# Autodesk Inventor assembly: Z Axis
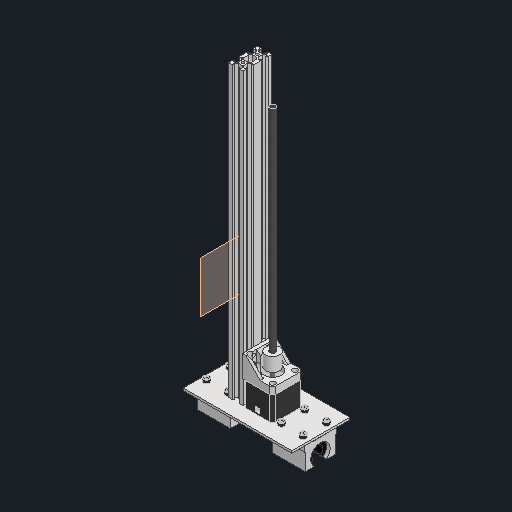
[picture p0: Inventor's stored thumbnail of the model, 512x512]
Saved by Autodesk Inventor 2025.1 (Build 291241000, 241)
## iProperties
Created: 2025-01-21
Part Number: Z Axis
Document SubType Name: Assembly
Designer: jerem
Author: jerem
## Documents named in this file (10)
- C:\Users\jerem\Documents\GitHub\Perovskite-Automated-Synthesis-System\CAD\Gantry\Z Axis.iam
- C:\Users\jerem\Documents\GitHub\Perovskite-Automated-Synthesis-System\CAD\Non 3D Printed Parts\X Axis Base Plate.ipt
- C:\Users\jerem\Documents\GitHub\Perovskite-Automated-Synthesis-System\CAD\Non 3D Printed Parts\Extrusion\V Extrustion 40x400mm.ipt
- C:\Users\jerem\Documents\GitHub\Perovskite-Automated-Synthesis-System\CAD\Non 3D Printed Parts\Screws\M5x12.ipt
- C:\Users\jerem\Documents\GitHub\Perovskite-Automated-Synthesis-System\CAD\Non 3D Printed Parts\Motors and Servos\NEMA17 Stepper Motor.ipt
- C:\Users\jerem\Documents\GitHub\Perovskite-Automated-Synthesis-System\CAD\Non 3D Printed Parts\Threaded Rod 300mm.ipt
- C:\Users\jerem\Documents\GitHub\Perovskite-Automated-Synthesis-System\CAD\Non 3D Printed Parts\Rod Coupler.ipt
- C:\Users\jerem\Documents\GitHub\Perovskite-Automated-Synthesis-System\CAD\Non 3D Printed Parts\Nuts\M4 T-Slot Nut.ipt
- C:\Users\jerem\Documents\GitHub\Perovskite-Automated-Synthesis-System\CAD\Gantry\Z Axis Motor Mount.ipt
- C:\Users\jerem\Documents\GitHub\Perovskite-Automated-Synthesis-System\CAD\Non 3D Printed Parts\Linear Rails\Linear Rail Slider Block.ipt
## Components (18 placed, 9 different names)
1. X Axis Base Plate:1 — Mate:1, Mate:2, Mate:3, Mate:4, Mate:5, Mate:6, Mate:7, Mate:8, Mate:9, Mate:10, Mate:11, Mate:12, Mate:13, Mate:14, Mate:15, Mate:16, Mate:17, Mate:26, Angle:1, Flush:2, Mate:42, Mate:43
2. V Extrustion 40x400mm:1 — Mate:1, Mate:25, Angle:1, Mate:30, Angle:2, Angle:3, Mate:32, Flush:1, Tangent:1
3. M5x12:1 — Mate:2, Mate:3, Mate:47
4. M5x12:2 — Mate:4, Mate:17
5. M5x12:3 — Mate:9, Mate:12
6. M5x12:4 — Mate:8, Mate:13
7. M5x12:5 — Mate:7, Mate:15, Tangent:1
8. M5x12:6 — Mate:6, Mate:14, Mate:45
9. M5x12:7 — Mate:5, Mate:16, Mate:46
10. M5x12:8 — Mate:10, Mate:11, Mate:44
11. NEMA17 Stepper Motor:1 — Mate:25, Mate:26, Mate:33, Mate:34, Mate:35, Flush:1, Flush:2
12. Threaded Rod 300mm:1
13. Rod Coupler:1
14. M4 T-Slot Nut:1 — Mate:30, Angle:2, Mate:37
15. M4 T-Slot Nut:2 — Angle:3, Mate:32, Mate:36
16. Z Axis Motor Mount:1 — Mate:33, Mate:34, Mate:35, Mate:36, Mate:37
17. Linear Rail Slider Block:1 — Mate:43, Mate:44, Mate:45
18. Linear Rail Slider Block:2 — Mate:42, Mate:46, Mate:47
## Relationships (42: Mate 36, Angle 3, Flush 2, Tangent 1)
- Mate:1: X Axis Base Plate:1 ↔ V Extrustion 40x400mm:1
- Mate:2: X Axis Base Plate:1 ↔ M5x12:1
- Mate:3: X Axis Base Plate:1 ↔ M5x12:1
- Mate:4: X Axis Base Plate:1 ↔ M5x12:2
- Mate:5: X Axis Base Plate:1 ↔ M5x12:7
- Mate:6: X Axis Base Plate:1 ↔ M5x12:6
- Mate:7: X Axis Base Plate:1 ↔ M5x12:5
- Mate:8: X Axis Base Plate:1 ↔ M5x12:4
- Mate:9: X Axis Base Plate:1 ↔ M5x12:3
- Mate:10: X Axis Base Plate:1 ↔ M5x12:8
- Mate:11: X Axis Base Plate:1 ↔ M5x12:8
- Mate:12: X Axis Base Plate:1 ↔ M5x12:3
- Mate:13: X Axis Base Plate:1 ↔ M5x12:4
- Mate:14: X Axis Base Plate:1 ↔ M5x12:6
- Mate:15: X Axis Base Plate:1 ↔ M5x12:5
- Mate:16: X Axis Base Plate:1 ↔ M5x12:7
- Mate:17: X Axis Base Plate:1 ↔ M5x12:2
- [Mate]: NEMA17 Stepper Motor:1 ↔ Rod Coupler:1
- [Mate]: Threaded Rod 300mm:1 ↔ Rod Coupler:1
- [Mate] (-8 mm): NEMA17 Stepper Motor:1 ↔ Rod Coupler:1
- [Mate] (-8 mm): Threaded Rod 300mm:1 ↔ Rod Coupler:1
- Mate:25: V Extrustion 40x400mm:1 ↔ NEMA17 Stepper Motor:1
- Mate:26: X Axis Base Plate:1 ↔ NEMA17 Stepper Motor:1
- Angle:1 (0 deg): X Axis Base Plate:1 ↔ V Extrustion 40x400mm:1
- Mate:30: V Extrustion 40x400mm:1 ↔ M4 T-Slot Nut:1
- Angle:2 (0 deg): V Extrustion 40x400mm:1 ↔ M4 T-Slot Nut:1
- Angle:3 (0 deg): V Extrustion 40x400mm:1 ↔ M4 T-Slot Nut:2
- Mate:32: V Extrustion 40x400mm:1 ↔ M4 T-Slot Nut:2
- Mate:33: NEMA17 Stepper Motor:1 ↔ Z Axis Motor Mount:1
- Mate:34: NEMA17 Stepper Motor:1 ↔ Z Axis Motor Mount:1
- Mate:35: NEMA17 Stepper Motor:1 ↔ Z Axis Motor Mount:1
- Mate:36: M4 T-Slot Nut:2 ↔ Z Axis Motor Mount:1
- Mate:37: M4 T-Slot Nut:1 ↔ Z Axis Motor Mount:1
- Flush:1: V Extrustion 40x400mm:1 ↔ NEMA17 Stepper Motor:1
- Flush:2: X Axis Base Plate:1 ↔ NEMA17 Stepper Motor:1
- Tangent:1: V Extrustion 40x400mm:1 ↔ M5x12:5
- Mate:42: X Axis Base Plate:1 ↔ Linear Rail Slider Block:2
- Mate:43: X Axis Base Plate:1 ↔ Linear Rail Slider Block:1
- Mate:44: M5x12:8 ↔ Linear Rail Slider Block:1
- Mate:45: M5x12:6 ↔ Linear Rail Slider Block:1
- Mate:46: M5x12:7 ↔ Linear Rail Slider Block:2
- Mate:47: M5x12:1 ↔ Linear Rail Slider Block:2
